# Autodesk Inventor assembly: AluM-StarS_MIR5
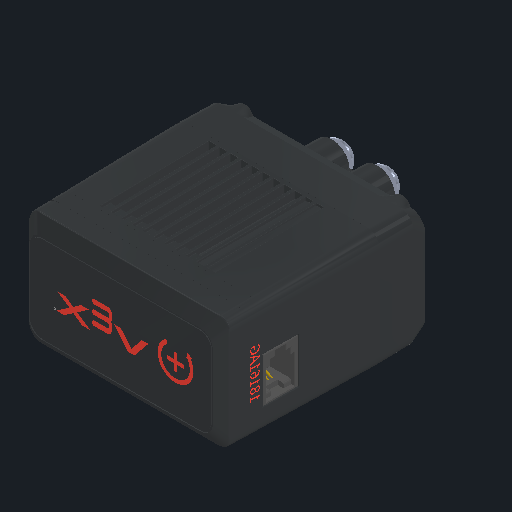
[picture p0: Inventor's stored thumbnail of the model, 512x512]
Saved by Autodesk Inventor 2024 (Build 280153000, 153)
## iProperties
Created: 2022-08-18
Part Number: AluM-StarS_MIR5
Document SubType Name: Assembly
Designer: macbook
Author: ylu12
## Documents named in this file (4)
- \\Mac\Home\Desktop\code\1599V-VRC\Cad\Electronics\Motors with Screws\AluM-StarS_MIR5.iam
- \\Mac\Home\Desktop\code\1599V-VRC\Cad\Electronics\V5 Motor_MIR5.ipt
- \\Mac\Home\Desktop\code\1599V-VRC\Cad\Structure\Hardware\Screw Steel - Star\SScrew Star Smooth .500.ipt
- \\Mac\Home\Desktop\code\1599V-VRC\Cad\Structure\Hardware\Screw Steel - Star.ipt
## Components (3 placed, 2 different names)
1. V5 Motor_MIR5:1
2. SScrew Star Smooth .500:1
3. SScrew Star Smooth .500:2
## Named parameters: Thickness = 1.6002 mm
